# Autodesk Inventor assembly: Hinge_V1_assembly
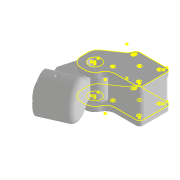
[picture p0: Inventor's stored thumbnail of the model, 180x180]
Saved by Autodesk Inventor 2022 (Build 260153000, 153)
## iProperties
Created: 2022-07-09
Part Number: Hinge_V1_assembly
Document SubType Name: Assembly
Designer: dell
Author: dell
## Documents named in this file (3)
- D:\xxxx\Uni\Part IV\MECHENG_700\Part_IV_project_CAD\Bird_skeleton_prototypes\Wing_drone_V1\Bird_wing_V2\Hinge_V1_assembly.iam
- D:\xxxx\Uni\Part IV\MECHENG_700\Part_IV_project_CAD\Bird_skeleton_prototypes\Wing_drone_V1\Bird_wing_V2\Hinge_p2.ipt
- D:\xxxx\Uni\Part IV\MECHENG_700\Part_IV_project_CAD\Bird_skeleton_prototypes\Wing_drone_V1\Bird_wing_V2\Hinge_p1_assembly.iam
## Components (2 placed, 2 different names)
1. Hinge_p2:1 — Mate:1, Mate:2
2. Hinge_p1_assembly:1 [sub-assembly] — Mate:1, Mate:2
## Relationships (2: Mate 2)
- Mate:1: Hinge_p2:1 ↔ Hinge_p1_assembly:1
- Mate:2 (0.1 mm): Hinge_p2:1 ↔ Hinge_p1_assembly:1
